# Autodesk Inventor assembly: Rb PEEK
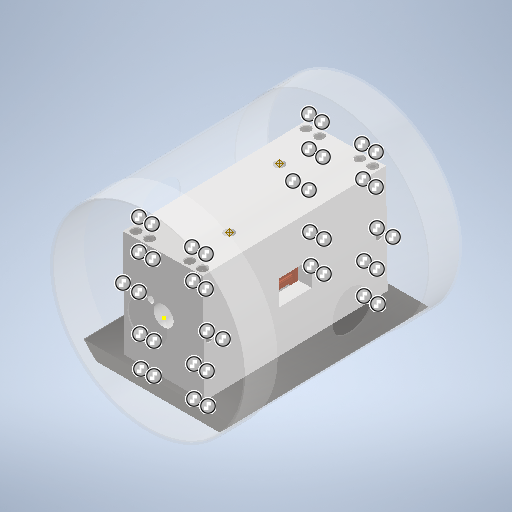
[picture p0: Inventor's stored thumbnail of the model, 512x512]
Saved by Autodesk Inventor 2025.3 (Build 293356000, 356)
## iProperties
Created: 2025-05-09
Part Number: Rb PEEK
Document SubType Name: Assembly
Designer: E. Moreno
Author: E. Moreno
Title: Rb PEEK - Ensamblado
## Documents named in this file (16)
- E:\Users\USER\Documents\GitHub\LAFriOC\Rb oven\Rb PEEK\Rb Full Modificación.iam
- E:\Users\USER\Documents\GitHub\LAFriOC\Rb oven\Rb PEEK\Rb PEEK - Arriba.ipt
- E:\Users\USER\Documents\GitHub\LAFriOC\Rb oven\Rb PEEK\Rb PEEK - Largo.ipt
- E:\Users\USER\Documents\GitHub\LAFriOC\Rb oven\Rb PEEK\Rb PEEK - Corto con ventana.ipt
- E:\Users\USER\Documents\GitHub\LAFriOC\Rb oven\Rb PEEK\Rb PEEK - Soporte.ipt
- E:\Users\USER\Documents\GitHub\LAFriOC\Rb oven\Rb PEEK\Rb PEEK - Abajo.ipt
- E:\Users\USER\Documents\GitHub\LAFriOC\Rb oven\Rb components\Cell.ipt
- E:\Users\USER\Documents\Inventor\Content Center Files\R2025\en-US\AS 1420\AS 1420 - 1973 - M4 x 25.ipt
- E:\Users\USER\Documents\Inventor\Content Center Files\R2025\en-US\AS 1420\AS 1420 - 1973 - M4 x 12.ipt
- E:\Users\USER\Documents\GitHub\LAFriOC\Rb oven\MS-1L Shield\Shield.iam
- E:\Users\USER\Documents\Inventor\Content Center Files\R2025\en-US\AS 1420\AS 1420 - 1973 - M6 x 16.ipt
- E:\Users\USER\Documents\GitHub\LAFriOC\Rb oven\Rb PEEK\Rb PEEK - Largo_MIR.ipt
- E:\Users\USER\Documents\GitHub\LAFriOC\Rb oven\Rb components\Thermistor.ipt
- E:\Users\USER\Documents\GitHub\LAFriOC\Rb oven\Rb housing\Rb oven housing - Bottom.iam
- E:\Users\USER\Documents\GitHub\LAFriOC\Rb oven\Rb housing\Rb oven housing - Top.iam
- E:\Users\USER\Documents\GitHub\LAFriOC\Rb oven\Rb components\Heater1-4.ipt
## Components (44 placed, 15 different names)
1. Shield:1 [sub-assembly] — Mate:41
2. Rb PEEK - Arriba:1 — Mate:1, Mate:2, Mate:3, Mate:5, Mate:6, Mate:33, Insert:9, Insert:10, Insert:11, Insert:12, Insert:13, Insert:14, Insert:15, Insert:16
3. Rb PEEK - Abajo:1 — Mate:21, Mate:22, Mate:23, Mate:29, Mate:30, Mate:34, Insert:21, Insert:24, Insert:25, Insert:26, Insert:27, Insert:28, Insert:29, Insert:30, Insert:33, Insert:34, Mate:38, Mate:39, Mate:41, Mate:44, Mate:45, Insert:46, Insert:47
4. Rb PEEK - Largo:1 — Mate:1, Mate:2, Mate:3, Mate:4, Mate:18, Mate:20, Mate:21, Mate:22, Mate:23, Insert:17, Insert:18
5. Rb PEEK - Largo_MIR:1 — Mate:38, Mate:39, Insert:44, Insert:45
6. Rb PEEK - Corto con ventana:1 — Mate:4, Mate:5, Mate:6
7. Rb PEEK - Corto con ventana:2 — Mate:18, Mate:20, Mate:33, Mate:34
8. Rb PEEK - Soporte:1 — Mate:29, Mate:45, Mate:46
9. Rb PEEK - Soporte:2 — Mate:30, Mate:44
10. Cell:1 — Mate:43
11. Rb oven housing - Top:1 [sub-assembly] — Insert:38, Insert:39, Insert:40, Insert:41, Mate:42
12. Rb oven housing - Bottom:1 [sub-assembly] — Insert:42, Insert:43, Mate:42, Mate:43, Mate:46
13. Thermistor:1 — Mate:47
14. Thermistor:2
15. Heater1-4:1 — Insert:43, Mate:47
16. Heater1-4:2 — Insert:42
17. AS 1420 - Metric M4 x 25:21 — Insert:38
18. AS 1420 - Metric M4 x 25:22 — Insert:39
19. AS 1420 - Metric M4 x 25:23 — Insert:40
20. AS 1420 - Metric M4 x 25:24 — Insert:41
21. AS 1420 - Metric M6 x 16:1 — Insert:33
22. AS 1420 - Metric M6 x 16:2 — Insert:34
23. AS 1420 - Metric M4 x 25:5 — Insert:9
24. AS 1420 - Metric M4 x 25:6 — Insert:10
25. AS 1420 - Metric M4 x 25:7 — Insert:11
26. AS 1420 - Metric M4 x 25:8 — Insert:12
27. AS 1420 - Metric M4 x 25:9 — Insert:13
28. AS 1420 - Metric M4 x 25:10 — Insert:14
29. AS 1420 - Metric M4 x 25:11 — Insert:15
30. AS 1420 - Metric M4 x 25:12 — Insert:16
31. AS 1420 - Metric M4 x 12:3 — Insert:17
32. AS 1420 - Metric M4 x 12:4 — Insert:18
33. AS 1420 - Metric M4 x 12:5 — Insert:44
34. AS 1420 - Metric M4 x 12:6 — Insert:45
35. AS 1420 - Metric M4 x 25:13 — Insert:21
36. AS 1420 - Metric M4 x 25:14 — Insert:24
37. AS 1420 - Metric M4 x 25:15 — Insert:25
38. AS 1420 - Metric M4 x 25:16 — Insert:26
39. AS 1420 - Metric M4 x 25:17 — Insert:27
40. AS 1420 - Metric M4 x 25:18 — Insert:28
41. AS 1420 - Metric M4 x 25:19 — Insert:29
42. AS 1420 - Metric M4 x 25:20 — Insert:30
43. AS 1420 - Metric M4 x 12:7 — Insert:46
44. AS 1420 - Metric M4 x 12:8 — Insert:47
## Relationships (54: Insert 30, Mate 24)
- Mate:1: Rb PEEK - Arriba:1 ↔ Rb PEEK - Largo:1
- Mate:2: Rb PEEK - Arriba:1 ↔ Rb PEEK - Largo:1
- Mate:3: Rb PEEK - Arriba:1 ↔ Rb PEEK - Largo:1
- Mate:4: Rb PEEK - Largo:1 ↔ Rb PEEK - Corto con ventana:1
- Mate:5: Rb PEEK - Arriba:1 ↔ Rb PEEK - Corto con ventana:1
- Mate:6: Rb PEEK - Arriba:1 ↔ Rb PEEK - Corto con ventana:1
- Mate:18: Rb PEEK - Largo:1 ↔ Rb PEEK - Corto con ventana:2
- Mate:20: Rb PEEK - Largo:1 ↔ Rb PEEK - Corto con ventana:2
- Mate:21: Rb PEEK - Abajo:1 ↔ Rb PEEK - Largo:1
- Mate:22: Rb PEEK - Abajo:1 ↔ Rb PEEK - Largo:1
- Mate:23: Rb PEEK - Abajo:1 ↔ Rb PEEK - Largo:1
- Mate:29: Rb PEEK - Abajo:1 ↔ Rb PEEK - Soporte:1
- Mate:30: Rb PEEK - Abajo:1 ↔ Rb PEEK - Soporte:2
- Mate:33: Rb PEEK - Arriba:1 ↔ Rb PEEK - Corto con ventana:2
- Mate:34: Rb PEEK - Abajo:1 ↔ Rb PEEK - Corto con ventana:2
- Insert:9: Rb PEEK - Arriba:1 ↔ AS 1420 - Metric M4 x 25:5
- Insert:10: Rb PEEK - Arriba:1 ↔ AS 1420 - Metric M4 x 25:6
- Insert:11: Rb PEEK - Arriba:1 ↔ AS 1420 - Metric M4 x 25:7
- Insert:12: Rb PEEK - Arriba:1 ↔ AS 1420 - Metric M4 x 25:8
- Insert:13: Rb PEEK - Arriba:1 ↔ AS 1420 - Metric M4 x 25:9
- Insert:14: Rb PEEK - Arriba:1 ↔ AS 1420 - Metric M4 x 25:10
- Insert:15: Rb PEEK - Arriba:1 ↔ AS 1420 - Metric M4 x 25:11
- Insert:16: Rb PEEK - Arriba:1 ↔ AS 1420 - Metric M4 x 25:12
- Insert:17: Rb PEEK - Largo:1 ↔ AS 1420 - Metric M4 x 12:3
- Insert:18: Rb PEEK - Largo:1 ↔ AS 1420 - Metric M4 x 12:4
- Insert:21: Rb PEEK - Abajo:1 ↔ AS 1420 - Metric M4 x 25:13
- Insert:24: Rb PEEK - Abajo:1 ↔ AS 1420 - Metric M4 x 25:14
- Insert:25: Rb PEEK - Abajo:1 ↔ AS 1420 - Metric M4 x 25:15
- Insert:26: Rb PEEK - Abajo:1 ↔ AS 1420 - Metric M4 x 25:16
- Insert:27: Rb PEEK - Abajo:1 ↔ AS 1420 - Metric M4 x 25:17
- Insert:28: Rb PEEK - Abajo:1 ↔ AS 1420 - Metric M4 x 25:18
- Insert:29: Rb PEEK - Abajo:1 ↔ AS 1420 - Metric M4 x 25:19
- Insert:30: Rb PEEK - Abajo:1 ↔ AS 1420 - Metric M4 x 25:20
- Insert:33: Rb PEEK - Abajo:1 ↔ AS 1420 - Metric M6 x 16:1
- Insert:34: Rb PEEK - Abajo:1 ↔ AS 1420 - Metric M6 x 16:2
- Mate:38: Rb PEEK - Abajo:1 ↔ Rb PEEK - Largo_MIR:1
- Mate:39: Rb PEEK - Abajo:1 ↔ Rb PEEK - Largo_MIR:1
- Mate:41: Shield:1 ↔ Rb PEEK - Abajo:1
- Insert:38: Rb oven housing - Top:1 ↔ AS 1420 - Metric M4 x 25:21
- Insert:39: Rb oven housing - Top:1 ↔ AS 1420 - Metric M4 x 25:22
- Insert:40: Rb oven housing - Top:1 ↔ AS 1420 - Metric M4 x 25:23
- Insert:41: Rb oven housing - Top:1 ↔ AS 1420 - Metric M4 x 25:24
- Insert:42 (-10.5 mm): Rb oven housing - Bottom:1 ↔ Heater1-4:2
- Insert:43 (-10.5 mm): Rb oven housing - Bottom:1 ↔ Heater1-4:1
- Mate:42: Rb oven housing - Top:1 ↔ Rb oven housing - Bottom:1
- Mate:43: Cell:1 ↔ Rb oven housing - Bottom:1
- Mate:44: Rb PEEK - Abajo:1 ↔ Rb PEEK - Soporte:2
- Mate:45: Rb PEEK - Abajo:1 ↔ Rb PEEK - Soporte:1
- Insert:44: Rb PEEK - Largo_MIR:1 ↔ AS 1420 - Metric M4 x 12:5
- Insert:45: Rb PEEK - Largo_MIR:1 ↔ AS 1420 - Metric M4 x 12:6
- Insert:46: Rb PEEK - Abajo:1 ↔ AS 1420 - Metric M4 x 12:7
- Insert:47: Rb PEEK - Abajo:1 ↔ AS 1420 - Metric M4 x 12:8
- Mate:46: Rb PEEK - Soporte:1 ↔ Rb oven housing - Bottom:1
- Mate:47 (-4.3 mm): Thermistor:1 ↔ Heater1-4:1
